# Autodesk Inventor assembly: omnicam_ass
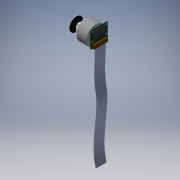
[picture p0: Inventor's stored thumbnail of the model, 180x180]
Saved by Autodesk Inventor 2017 (Build 210142000, 142)
## iProperties
Created: 2018-05-10
Part Number: omnicam_ass
Document SubType Name: Assembly
Designer: Nic
Author: Nic
## Documents named in this file (6)
- C:\Users\Nic\Documents\iDripper\omnicam_ass.iam
- C:\Users\Nic\Documents\iDripper\omnicam.ipt
- C:\Users\Nic\Documents\iDripper\mirror_support.ipt
- C:\Users\Nic\Documents\iDripper\omni_mirror.ipt
- C:\Users\Nic\Documents\iDripper\omnilens.ipt
- C:\Users\Nic\Documents\iDripper\RasPi_Camera.iam
## Components (5 placed, 5 different names)
1. omnicam:1 — Insert:1, Insert:3, Insert:4
2. mirror_support:1 — Insert:1, Insert:2
3. omni_mirror:1 — Insert:2
4. omnilens:1 — Insert:3
5. RasPi_Camera:1 [sub-assembly] — Insert:4
## Relationships (4: Insert 4)
- Insert:1: omnicam:1 ↔ mirror_support:1
- Insert:2: mirror_support:1 ↔ omni_mirror:1
- Insert:3: omnicam:1 ↔ omnilens:1
- Insert:4: omnicam:1 ↔ RasPi_Camera:1
